# Autodesk Inventor assembly: multi-spindle
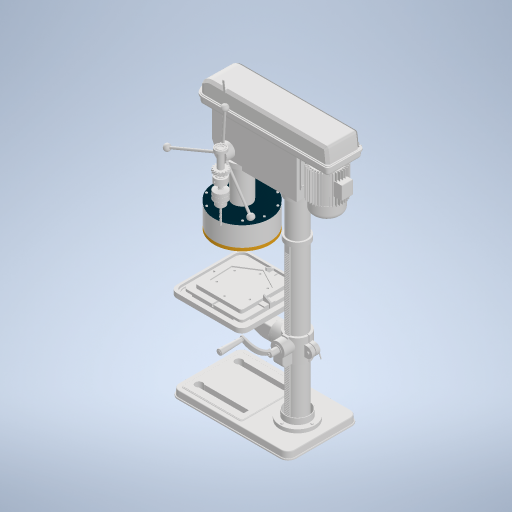
[picture p0: Inventor's stored thumbnail of the model, 512x512]
Saved by Autodesk Inventor 2024.2 (Build 282272000, 272)
## iProperties
Created: 2021-09-13
Part Number: multi-spindle
Description: STEP AP203
Document SubType Name: Assembly
Designer: 062210026
Title: multi-spindle.STEP
Author: Moghimi
Revision Number: ANY
Sending System: SolidWorks 2018
Preprocessor: SwSTEP 2.0
## Documents named in this file (37)
- C:\Users\062210026\Desktop\ProjInt3\Maquina\multi-spindle.iam
- C:\Users\062210026\Desktop\NX\multi-spindle\1_Varsay_lan.ipt
- C:\Users\062210026\Desktop\NX\multi-spindle\2_Varsay_lan.ipt
- C:\Users\062210026\Desktop\NX\multi-spindle\4_Varsay_lan.ipt
- C:\Users\062210026\Desktop\NX\multi-spindle\5_Varsay_lan.ipt
- C:\Users\062210026\Desktop\NX\multi-spindle\6_Varsay_lan.ipt
- C:\Users\062210026\Desktop\NX\multi-spindle\7_Varsay_lan.ipt
- C:\Users\062210026\Desktop\NX\multi-spindle\8_Varsay_lan.ipt
- C:\Users\062210026\Desktop\NX\multi-spindle\9_Varsay_lan.ipt
- C:\Users\062210026\Desktop\NX\multi-spindle\10_Varsay_lan.ipt
- C:\Users\062210026\Desktop\NX\multi-spindle\11_Varsay_lan.ipt
- C:\Users\062210026\Desktop\NX\multi-spindle\12_Varsay_lan.ipt
- C:\Users\062210026\Desktop\NX\multi-spindle\13_Varsay_lan.ipt
- C:\Users\062210026\Desktop\NX\multi-spindle\14_Varsay_lan.ipt
- C:\Users\062210026\Desktop\NX\multi-spindle\15_Varsay_lan.ipt
- C:\Users\062210026\Desktop\NX\multi-spindle\16_Varsay_lan.ipt
- C:\Users\062210026\Desktop\NX\multi-spindle\hex bolt gradeab_iso_ISO 4014 - M4 x 35 x 14-N.ipt
- C:\Users\062210026\Desktop\NX\multi-spindle\hex bolt gradeab_iso_ISO 4014 - M3 x 20 x 12-N.ipt
- C:\Users\062210026\Desktop\NX\multi-spindle\hex bolt gradeab_iso_ISO 4014 - M6 x 30 x 18-N.ipt
- C:\Users\062210026\Desktop\NX\multi-spindle\slotted cheese head screw_iso_ISO 1207 - M6 x 8 - 8N.ipt
- C:\Users\062210026\Desktop\NX\multi-spindle\SKF_6004.iam
- C:\Users\062210026\Desktop\NX\multi-spindle\MAILN AX.ipt
- C:\Users\062210026\Desktop\NX\multi-spindle\UPPER PLATE.ipt
- C:\Users\062210026\Desktop\NX\multi-spindle\SKF_30204.iam
- C:\Users\062210026\Desktop\NX\multi-spindle\helical gear_3_am2_Metric - RH Helical gear 2.5M 30T 45HA 20PA 15FW ---30N75H50L35.0R1.ipt
- C:\Users\062210026\Desktop\NX\multi-spindle\6-AX.ipt
- C:\Users\062210026\Desktop\NX\multi-spindle\helical gear_3_am2_Metric - RH Helical gear 2.5M 15T 45HA 20PA 15FW ---15N75H50L25.0R1.ipt
- C:\Users\062210026\Desktop\NX\multi-spindle\SHEL.ipt
- C:\Users\062210026\Desktop\NX\multi-spindle\socket head cap screw_am_B18.3.1M - 5 x 0.8 x 20 Hex SHCS -- 20NHX.ipt
- C:\Users\062210026\Desktop\NX\multi-spindle\STRIGHTER.ipt
- C:\Users\062210026\Desktop\NX\multi-spindle\KEY.ipt
- C:\Users\062210026\Desktop\NX\multi-spindle\spring pin slotted_ai_SPS 0.25x1.25.ipt
- C:\Users\062210026\Desktop\NX\multi-spindle\socket head cap screw_am_B18.3.1M - 5 x 0.8 x 30 Hex SHCS -- 22NHX.ipt
- C:\Users\062210026\Desktop\NX\multi-spindle\Drill.ipt
- C:\Users\062210026\Desktop\NX\multi-spindle\FIXTURE.ipt
- C:\Users\062210026\Desktop\NX\multi-spindle\WORKPICE.ipt
- C:\Users\062210026\Desktop\TampaBaixoFuras\TampaBaixo.ipt
## Components (87 placed, 78 different names)
1. SKF_30204:7 [sub-assembly]
2. helical gear_3_am2_Metric - RH Helical gear 2.5M 15T 45HA 20PA 15FW ---15N75H50L25.0R1:7
3. 6-AX:7
4. spring pin slotted_ai_SPS 0.25x1.25:7
5. 15_Varsay_lan:8
6. Drill:7
7. 1_Varsay_lan_1
8. 2_Varsay_lan_2
9. 4_Varsay_lan_3
10. 5_Varsay_lan_4
11. 6_Varsay_lan_5
12. 7_Varsay_lan_6
13. 8_Varsay_lan_7
14. 9_Varsay_lan_8
15. 10_Varsay_lan_9
16. 11_Varsay_lan_10
17. 12_Varsay_lan_11
18. 13_Varsay_lan_12
19. 14_Varsay_lan_13
20. 14_Varsay_lan_14
21. 14_Varsay_lan_15
22. 15_Varsay_lan_16
23. 16_Varsay_lan_17
24. 16_Varsay_lan_18
25. hex bolt gradeab_iso_ISO 4014 - M4 x 35 x 14-N_19
26. hex bolt gradeab_iso_ISO 4014 - M4 x 35 x 14-N_20
27. hex bolt gradeab_iso_ISO 4014 - M4 x 35 x 14-N_21
28. hex bolt gradeab_iso_ISO 4014 - M4 x 35 x 14-N_22
29. hex bolt gradeab_iso_ISO 4014 - M3 x 20 x 12-N_23
30. hex bolt gradeab_iso_ISO 4014 - M3 x 20 x 12-N_24
31. hex bolt gradeab_iso_ISO 4014 - M3 x 20 x 12-N_25
32. hex bolt gradeab_iso_ISO 4014 - M3 x 20 x 12-N_26
33. hex bolt gradeab_iso_ISO 4014 - M6 x 30 x 18-N_27
34. hex bolt gradeab_iso_ISO 4014 - M6 x 30 x 18-N_28
35. hex bolt gradeab_iso_ISO 4014 - M6 x 30 x 18-N_29
36. hex bolt gradeab_iso_ISO 4014 - M6 x 30 x 18-N_30
37. hex bolt gradeab_iso_ISO 4014 - M6 x 30 x 18-N_31
38. slotted cheese head screw_iso_ISO 1207 - M6 x 8 - 8N_32
39. SKF_6004_34 [sub-assembly]
40. SKF_6004_35 [sub-assembly] — Mate:1
41. MAILN AX_36
42. UPPER PLATE_37
43. SKF_6004_39 [sub-assembly]
44. helical gear_3_am2_Metric - RH Helical gear 2.5M 30T 45HA 20PA 15FW ---30N75H50L35.0R1_40
45. SHEL_43
46. socket head cap screw_am_B18.3.1M - 5 x 0.8 x 20 Hex SHCS -- 20NHX_44
47. STRIGHTER_46
48. KEY_47
49. SKF_6004_50 [sub-assembly]
50. SKF_6004_52 [sub-assembly]
51. SKF_6004_53 [sub-assembly]
52. SKF_6004_54 [sub-assembly]
53. helical gear_3_am2_Metric - RH Helical gear 2.5M 15T 45HA 20PA 15FW ---15N75H50L25.0R1_60
54. helical gear_3_am2_Metric - RH Helical gear 2.5M 15T 45HA 20PA 15FW ---15N75H50L25.0R1_61
55. helical gear_3_am2_Metric - RH Helical gear 2.5M 15T 45HA 20PA 15FW ---15N75H50L25.0R1_62
56. helical gear_3_am2_Metric - RH Helical gear 2.5M 15T 45HA 20PA 15FW ---15N75H50L25.0R1_63
57. helical gear_3_am2_Metric - RH Helical gear 2.5M 15T 45HA 20PA 15FW ---15N75H50L25.0R1_64
58. socket head cap screw_am_B18.3.1M - 5 x 0.8 x 20 Hex SHCS -- 20NHX_70
59. socket head cap screw_am_B18.3.1M - 5 x 0.8 x 20 Hex SHCS -- 20NHX_71
60. socket head cap screw_am_B18.3.1M - 5 x 0.8 x 20 Hex SHCS -- 20NHX_72
61. socket head cap screw_am_B18.3.1M - 5 x 0.8 x 20 Hex SHCS -- 20NHX_73
62. socket head cap screw_am_B18.3.1M - 5 x 0.8 x 20 Hex SHCS -- 20NHX_75
63. socket head cap screw_am_B18.3.1M - 5 x 0.8 x 20 Hex SHCS -- 20NHX_76
64. socket head cap screw_am_B18.3.1M - 5 x 0.8 x 20 Hex SHCS -- 20NHX_77
65. socket head cap screw_am_B18.3.1M - 5 x 0.8 x 20 Hex SHCS -- 20NHX_78
66. socket head cap screw_am_B18.3.1M - 5 x 0.8 x 30 Hex SHCS -- 22NHX_98
67. socket head cap screw_am_B18.3.1M - 5 x 0.8 x 30 Hex SHCS -- 22NHX_99
68. socket head cap screw_am_B18.3.1M - 5 x 0.8 x 30 Hex SHCS -- 22NHX_100
69. socket head cap screw_am_B18.3.1M - 5 x 0.8 x 30 Hex SHCS -- 22NHX_101
70. socket head cap screw_am_B18.3.1M - 5 x 0.8 x 30 Hex SHCS -- 22NHX_102
71. socket head cap screw_am_B18.3.1M - 5 x 0.8 x 30 Hex SHCS -- 22NHX_103
72. socket head cap screw_am_B18.3.1M - 5 x 0.8 x 30 Hex SHCS -- 22NHX_104
73. FIXTURE_111
74. FIXTURE_112
75. WORKPICE_113
76. TampaBaixo:1 — Mate:1, Mate:3, Mate:4, Mate:5, Mate:6, Mate:7, Mate:8, Mate:9, Mate:10, Mate:11
77. socket head cap screw_am_B18.3.1M - 5 x 0.8 x 20 Hex SHCS -- 20NHX:21 — Mate:3
78. socket head cap screw_am_B18.3.1M - 5 x 0.8 x 20 Hex SHCS -- 20NHX:22 — Mate:8
79. socket head cap screw_am_B18.3.1M - 5 x 0.8 x 20 Hex SHCS -- 20NHX:23 — Mate:10
80. socket head cap screw_am_B18.3.1M - 5 x 0.8 x 20 Hex SHCS -- 20NHX:24
81. socket head cap screw_am_B18.3.1M - 5 x 0.8 x 20 Hex SHCS -- 20NHX:26 — Mate:5
82. socket head cap screw_am_B18.3.1M - 5 x 0.8 x 20 Hex SHCS -- 20NHX:27 — Mate:6
83. socket head cap screw_am_B18.3.1M - 5 x 0.8 x 20 Hex SHCS -- 20NHX:28 — Mate:9
84. socket head cap screw_am_B18.3.1M - 5 x 0.8 x 20 Hex SHCS -- 20NHX:30 — Mate:11
85. socket head cap screw_am_B18.3.1M - 5 x 0.8 x 20 Hex SHCS -- 20NHX:32 — Mate:7
86. socket head cap screw_am_B18.3.1M - 5 x 0.8 x 20 Hex SHCS -- 20NHX:33 — Mate:4
87. socket head cap screw_am_B18.3.1M - 5 x 0.8 x 20 Hex SHCS -- 20NHX_74
## Relationships (10: Mate 10)
- Mate:1: SKF_6004_35 ↔ TampaBaixo:1
- Mate:3: TampaBaixo:1 ↔ socket head cap screw_am_B18.3.1M - 5 x 0.8 x 20 Hex SHCS -- 20NHX:21
- Mate:4: TampaBaixo:1 ↔ socket head cap screw_am_B18.3.1M - 5 x 0.8 x 20 Hex SHCS -- 20NHX:33
- Mate:5: TampaBaixo:1 ↔ socket head cap screw_am_B18.3.1M - 5 x 0.8 x 20 Hex SHCS -- 20NHX:26
- Mate:6: TampaBaixo:1 ↔ socket head cap screw_am_B18.3.1M - 5 x 0.8 x 20 Hex SHCS -- 20NHX:27
- Mate:7: TampaBaixo:1 ↔ socket head cap screw_am_B18.3.1M - 5 x 0.8 x 20 Hex SHCS -- 20NHX:32
- Mate:8: TampaBaixo:1 ↔ socket head cap screw_am_B18.3.1M - 5 x 0.8 x 20 Hex SHCS -- 20NHX:22
- Mate:9: TampaBaixo:1 ↔ socket head cap screw_am_B18.3.1M - 5 x 0.8 x 20 Hex SHCS -- 20NHX:28
- Mate:10: TampaBaixo:1 ↔ socket head cap screw_am_B18.3.1M - 5 x 0.8 x 20 Hex SHCS -- 20NHX:23
- Mate:11: TampaBaixo:1 ↔ socket head cap screw_am_B18.3.1M - 5 x 0.8 x 20 Hex SHCS -- 20NHX:30
